# Autodesk Inventor assembly: #SHOOTER.3
(part 2 of 2)
- Insert:139: PLATE,SHOOTER,BOTTOM:1 ↔ PURCHASED,M4x12mm,BUTTONHEAD,BOLT:3
- Insert:140: PLATE,SHOOTER,BOTTOM:1 ↔ PURCHASED,M4x12mm,BUTTONHEAD,BOLT:4
- Insert:141: PLATE,SHOOTER,BOTTOM:1 ↔ PURCHASED,M4x12mm,BUTTONHEAD,BOLT:5
- Insert:142: PLATE,SHOOTER,BOTTOM:1 ↔ PURCHASED,M4x12mm,BUTTONHEAD,BOLT:6
- Insert:143: PLATE,SHOOTER,BOTTOM:1 ↔ PURCHASED,M4x12mm,BUTTONHEAD,BOLT:7
- Insert:144: PLATE,SHOOTER,BOTTOM:1 ↔ PURCHASED,M4x12mm,BUTTONHEAD,BOLT:8
- Insert:145: PLATE,SHOOTER,SIDE:2 ↔ PURCHASED,0.25-20x0.5in,BUTTONHEAD,BOLT:4
- Insert:146: PLATE,SHOOTER,SIDE:1 ↔ PURCHASED,0.25-20x0.5in,BUTTONHEAD,BOLT:1
- Insert:151: PLATE,SHOOTER,BOTTOM:1 ↔ 3DPRINT,BACKRAIL_MIR:1
- Mate:137: PLATE,SHOOTER,BOTTOM:1 ↔ 3DPRINT,BACKRAIL_MIR:1
- Mate:138: PLATE,SHOOTER,SIDE:1 ↔ STANDIN,130T,HTD5mm,BELT:1
- Mate:139: PLATE,SHOOTER,SIDE:1 ↔ STANDIN,130T,HTD5mm,BELT:1
- Mate:140 (0.75 mm): PURCHASED,HTD5mm,24T,PULLEY:1 ↔ STANDIN,130T,HTD5mm,BELT:1
- Mate:141: STOCK,SHAFT,HEX,SHOOTER:1 ↔ PURCHASED,HTD5mm,20T,PULLEY:3
- Mate:142: STOCK,SHAFT,HEX,SHOOTER:1 ↔ PURCHASED,HTD5mm,20T,PULLEY:3
- Mate:144: STOCK,SHAFT,HEX,HOOD,REVERSER:1 ↔ PURCHASED,HTD5mm,20T,PULLEY:4
- Mate:145: STOCK,SHAFT,HEX,HOOD,REVERSER:1 ↔ PURCHASED,HTD5mm,20T,PULLEY:4
- Mate:146: PURCHASED,GEAR,20DP,30T,HEX:1 ↔ PURCHASED,HTD5mm,20T,PULLEY:4
- Rotation:1 [RelateRotation] (1 ul): STOCK,SHAFT,HEX,MOTORS:1 ↔ STOCK,SHAFT,HEX,SHOOTER:1
- Mate:147: PLATE,HOOD,SIDE:2 ↔ STANDIN,45T,HTD5mm,BELT:1
- Mate:148: PLATE,HOOD,SIDE:2 ↔ STANDIN,45T,HTD5mm,BELT:1
- Mate:149: PLATE,SHOOTER,SIDE:2 ↔ STANDIN,90T,HTD5mm,BELT:1
- Mate:150: PLATE,HOOD,SIDE:2 ↔ STANDIN,90T,HTD5mm,BELT:1
- Mate:151 (0.75 mm): PURCHASED,HTD5mm,20T,PULLEY:4 ↔ STANDIN,90T,HTD5mm,BELT:1
- Mate:152 (0.75 mm): PURCHASED,HTD5mm,20T,PULLEY:1 ↔ STANDIN,45T,HTD5mm,BELT:1
- Flush:9: STOCK,SHAFT,HEX,SHOOTER:1 ↔ PURCHASED,HTD5mm,20T,PULLEY:3
- Mate:153: STOCK,SHAFT,HEX,SHOOTER:1 ↔ 3DPRINT,FLYWHEELTOHOOD,SPACER:1
- Mate:154: STOCK,SHAFT,HEX,SHOOTER:1 ↔ 3DPRINT,FLYWHEELTOHOOD,SPACER:1
- Mate:155: PURCHASED,HEX_BEARING:9 ↔ 3DPRINT,FLYWHEELTOHOOD,SPACER:1
- Insert:152: PLATE,HOOD,SIDE:1 ↔ STOCK,HOOD,SPACER,10-32,6.25in:1
- Insert:153: PLATE,HOOD,SIDE:2 ↔ STOCK,HOOD,SPACER,10-32,6.25in:2
- Insert:154: PLATE,HOOD,SIDE:1 ↔ PURCHASED,10-32x0.5in,BUTTONHEAD,BOLT:49
- Insert:155: PLATE,HOOD,SIDE:1 ↔ PURCHASED,10-32x0.5in,BUTTONHEAD,BOLT:51
- Insert:156: PLATE,HOOD,SIDE:2 ↔ PURCHASED,10-32x0.5in,BUTTONHEAD,BOLT:50
- Insert:157: PLATE,HOOD,SIDE:2 ↔ PURCHASED,10-32x0.5in,BUTTONHEAD,BOLT:52
- Insert:158: PLATE,SHOOTER,BOTTOM:1 ↔ 3DPRINT,BACKRAIL:1
- Mate:156 (1.5977 mm): PURCHASED,HEX_BEARING:1 ↔ PURCHASED,HEX_BEARING:10
- Mate:157: STOCK,SHAFT,HEX,SHOOTER:1 ↔ 3DPRINT,SIDEPLATETOHOOD,SPACER :1
- Mate:158: STOCK,SHAFT,HEX,SHOOTER:1 ↔ 3DPRINT,SIDEPLATETOHOOD,SPACER :1
- Mate:159: PURCHASED,HEX_BEARING:11 ↔ 3DPRINT,SIDEPLATETOHOOD,SPACER :1
- Mate:160: STOCK,SHAFT,HEX,SHOOTER:1 ↔ 3DPRINT,SIDEPLATETOHOOD,SPACER :2
- Mate:161: STOCK,SHAFT,HEX,SHOOTER:1 ↔ 3DPRINT,SIDEPLATETOHOOD,SPACER :2
- Mate:162: PURCHASED,HEX_BEARING:10 ↔ 3DPRINT,SIDEPLATETOHOOD,SPACER :2
- Mate:163: PLATE.HOOD,PINION,GEAR:1 ↔ 3DPRINT,HOOD,DRIVEGEAR,SPACER:1
- Mate:164: STOCK,HEX,ROUND,HOOD:1 ↔ 3DPRINT,BUSHINGTOHOODDRIVEGEAR,SPACER:1
- Mate:165: STOCK,HEX,ROUND,HOOD:1 ↔ 3DPRINT,BUSHINGTOHOODDRIVEGEAR,SPACER:1
- Mate:166: PURCHASED,BUSHING,13.75mmID,0.75inOD:1 ↔ 3DPRINT,BUSHINGTOHOODDRIVEGEAR,SPACER:1
- Mate:167: PLATE.HOOD,PINION,GEAR:1 ↔ 3DPRINT,BUSHINGTOHOODDRIVEGEAR,SPACER:1
- Mate:168: STOCK,HEX,ROUND,HOOD:1 ↔ 3DPRINT,BUSHINGTOHOODDRIVEGEAR,SPACER:2
- Mate:169: STOCK,HEX,ROUND,HOOD:1 ↔ 3DPRINT,BUSHINGTOHOODDRIVEGEAR,SPACER:2
- Mate:170: PURCHASED,BUSHING,13.75mmID,0.75inOD:2 ↔ 3DPRINT,BUSHINGTOHOODDRIVEGEAR,SPACER:2
- Mate:171: STOCK,HEX,ROUND,HOOD:1 ↔ 3DPRINT,SIDEPLATETOHOODGEAR,SPACER:1
- Mate:172: STOCK,HEX,ROUND,HOOD:1 ↔ 3DPRINT,SIDEPLATETOHOODGEAR,SPACER:1
- Mate:173: PURCHASED,BUSHING,13.75mmID,0.75inOD:1 ↔ 3DPRINT,SIDEPLATETOHOODGEAR,SPACER:1
- Mate:174: PLATE,HOOD,SIDE:1 ↔ PLATE,SHOOTER,BOTTOM:1
- Insert:159: PLATE,SHOOTER,BACK:1 ↔ PLATE,NUTBLOCK,BACK:1
- Insert:160: PLATE,SHOOTER,BOTTOM:1 ↔ PLATE,NUTBLOCK,BACK:1
- Insert:161: PLATE,HOOD,SIDE:1 ↔ 3DPRINT,HOOD,ALIGNMENT,PLATES:1
- Insert:163: PLATE,HOOD,SIDE:1 ↔ 3DPRINT,HOOD,ALIGNMENT,PLATES:2
- Insert:164: PLATE,HOOD,SIDE:1 ↔ 3DPRINT,HOOD,ALIGNMENT,PLATES:2
- Insert:165: PLATE,HOOD,SIDE:1 ↔ 3DPRINT,HOOD,ALIGNMENT,PLATES:1
- Insert:166: PLATE,HOOD,SIDE:2 ↔ 3DPRINT,HOOD,ALIGNMENT,PLATES:3
- Insert:167: PLATE,HOOD,SIDE:2 ↔ 3DPRINT,HOOD,ALIGNMENT,PLATES:3
- Insert:168: PLATE,HOOD,SIDE:2 ↔ 3DPRINT,HOOD,ALIGNMENT,PLATES:4
- Insert:169: PLATE,HOOD,SIDE:2 ↔ 3DPRINT,HOOD,ALIGNMENT,PLATES:4
- Insert:170: 3DPRINT,HOOD,ALIGNMENT,PLATES:3 ↔ PURCHASED,M3x16mm,BUTTONHEAD,BOLT:1
- Insert:171: 3DPRINT,HOOD,ALIGNMENT,PLATES:3 ↔ PURCHASED,M3x16mm,BUTTONHEAD,BOLT:2
- Insert:172: 3DPRINT,HOOD,ALIGNMENT,PLATES:3 ↔ PURCHASED,M3x16mm,BUTTONHEAD,BOLT:3
- Insert:173: 3DPRINT,HOOD,ALIGNMENT,PLATES:3 ↔ PURCHASED,M3x16mm,BUTTONHEAD,BOLT:4
- Insert:174: 3DPRINT,HOOD,ALIGNMENT,PLATES:1 ↔ PURCHASED,M3x16mm,BUTTONHEAD,BOLT:5
- Insert:175: 3DPRINT,HOOD,ALIGNMENT,PLATES:1 ↔ PURCHASED,M3x16mm,BUTTONHEAD,BOLT:6
- Insert:176: 3DPRINT,HOOD,ALIGNMENT,PLATES:1 ↔ PURCHASED,M3x16mm,BUTTONHEAD,BOLT:7
- Insert:177: 3DPRINT,HOOD,ALIGNMENT,PLATES:1 ↔ PURCHASED,M3x16mm,BUTTONHEAD,BOLT:8
- Insert:178: 3DPRINT,HOOD,ALIGNMENT,PLATES:1 ↔ PURCHASED,M3x16mm,BUTTONHEAD,BOLT:9
- Insert:179: 3DPRINT,HOOD,ALIGNMENT,PLATES:2 ↔ PURCHASED,M3,NYLOCK,NUT:11
- Insert:180: 3DPRINT,HOOD,ALIGNMENT,PLATES:2 ↔ PURCHASED,M3,NYLOCK,NUT:10
- Insert:181: 3DPRINT,HOOD,ALIGNMENT,PLATES:2 ↔ PURCHASED,M3,NYLOCK,NUT:9
- Insert:182: 3DPRINT,HOOD,ALIGNMENT,PLATES:2 ↔ PURCHASED,M3,NYLOCK,NUT:8
- Insert:183: 3DPRINT,HOOD,ALIGNMENT,PLATES:2 ↔ PURCHASED,M3,NYLOCK,NUT:7
- Insert:184: 3DPRINT,HOOD,ALIGNMENT,PLATES:4 ↔ PURCHASED,M3,NYLOCK,NUT:6
- Insert:185: 3DPRINT,HOOD,ALIGNMENT,PLATES:4 ↔ PURCHASED,M3,NYLOCK,NUT:5
- Insert:186: 3DPRINT,HOOD,ALIGNMENT,PLATES:4 ↔ PURCHASED,M3,NYLOCK,NUT:1
- Insert:187: 3DPRINT,HOOD,ALIGNMENT,PLATES:4 ↔ PURCHASED,M3,NYLOCK,NUT:3
- Mate:181 (13.97 mm): PLATE,NUTBLOCK:4 ↔ 3DPRINT,LIMIT_SWITCH,SPACER:1
- Mate:182: PLATE,SHOOTER,SIDE:1 ↔ 3DPRINT,LIMIT_SWITCH,SPACER:1
- Mate:183: PLATE,SHOOTER,BOTTOM:1 ↔ 3DPRINT,LIMIT_SWITCH,SPACER:1
- Mate:184: CONTROLS,LIMIT_SWITCH,VEX:1 ↔ 3DPRINT,LIMIT_SWITCH,SPACER:1
- Mate:185: PLATE,SHOOTER,BOTTOM:1 ↔ CONTROLS,LIMIT_SWITCH,VEX:1
- Mate:186: CONTROLS,LIMIT_SWITCH,VEX:1 ↔ 3DPRINT,LIMIT_SWITCH,SPACER:1
- Mate:187: PLATE,SHOOTER,SIDE:1 ↔ PURCHASED,M4x12mm,BUTTONHEAD,BOLT:9
- Mate:188: CONTROLS,LIMIT_SWITCH,VEX:1 ↔ PURCHASED,M4x12mm,BUTTONHEAD,BOLT:9
- Mate:189: PLATE,SHOOTER,SIDE:1 ↔ PURCHASED,M4x12mm,BUTTONHEAD,BOLT:10
- Mate:190: CONTROLS,LIMIT_SWITCH,VEX:1 ↔ PURCHASED,M4x12mm,BUTTONHEAD,BOLT:10
